# Autodesk Inventor assembly: circuittmp
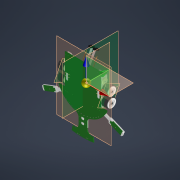
[picture p0: Inventor's stored thumbnail of the model, 180x180]
Saved by Autodesk Inventor 2022 (Build 260153000, 153)
## iProperties
Created: 2022-02-06
Part Number: circuittmp
Document SubType Name: Assembly
Designer: shiokaze
Author: shiokaze
## Documents named in this file (10)
- C:\Users\shiok\Documents\GitHub\murakumo\inventor\circuittmp.iam
- C:\Users\shiok\Documents\GitHub\murakumo\circuit\kicad\Step\Main.iam
- C:\Users\shiok\Documents\GitHub\murakumo\circuit\kicad\Step\Power.iam
- C:\Users\shiok\Documents\GitHub\murakumo\circuit\kicad\Step\SubSensor.iam
- C:\Users\shiok\Documents\GitHub\murakumo\circuit\kicad\Step\FrontSensor.iam
- C:\Users\shiok\Documents\GitHub\murakumo\inventor\Motor_MIR.iam
- C:\Users\shiok\Documents\GitHub\murakumo\inventor\jump.ipt
- C:\Users\shiok\Documents\GitHub\murakumo\inventor\SideSensorMount.ipt
- C:\Users\shiok\Documents\GitHub\murakumo\inventor\battery.ipt
- C:\Users\shiok\Documents\GitHub\murakumo\inventor\Motor_MIR_MIR.iam
## Components (11 placed, 9 different names)
1. Main:1 [sub-assembly] — メイト:1, メイト:2, メイト:3, メイト:10, 挿入:1, メイト:13, メイト:14, メイト:15, 角度:1, メイト:18, 挿入:2, メイト:25
2. Power:1 [sub-assembly] — メイト:4, メイト:5, メイト:6, 対称度:1, フラッシュ:1
3. SubSensor:2 [sub-assembly] — メイト:7, メイト:8, メイト:9
4. FrontSensor:1 [sub-assembly] — メイト:12, メイト:16, メイト:17
5. Motor_MIR:1 [sub-assembly] — メイト:1, メイト:2, メイト:3, メイト:4, メイト:5, メイト:6, 対称度:1, メイト:26
6. jump:1 — メイト:12, メイト:13, メイト:14, メイト:15, メイト:16, メイト:17
7. SideSensorMount:1 — メイト:7, メイト:8, メイト:9, メイト:10, 挿入:1
8. battery:1 — メイト:18, メイト:19, メイト:20
9. SideSensorMount:2 — メイト:21, メイト:22, メイト:23, 挿入:2
10. SubSensor:3 [sub-assembly] — メイト:21, メイト:22, メイト:23
11. Motor_MIR_MIR:1 [sub-assembly] — フラッシュ:2
## Relationships (31: Mate 25, Insert 2, Flush 2, Symmetry 1, Angle 1)
- メイト:1 [Mate]: Main:1 ↔ Motor_MIR:1
- メイト:2 [Mate]: Main:1 ↔ Motor_MIR:1
- メイト:3 [Mate]: Main:1 ↔ Motor_MIR:1
- メイト:4 [Mate]: Power:1 ↔ Motor_MIR:1
- メイト:5 [Mate]: Power:1 ↔ Motor_MIR:1
- メイト:6 [Mate]: Power:1 ↔ Motor_MIR:1
- 対称度:1 [Symmetry]: Power:1 ↔ Motor_MIR:1
- メイト:7 [Mate]: SubSensor:2 ↔ SideSensorMount:1
- メイト:8 [Mate]: SubSensor:2 ↔ SideSensorMount:1
- メイト:9 [Mate]: SubSensor:2 ↔ SideSensorMount:1
- メイト:10 [Mate]: Main:1 ↔ SideSensorMount:1
- 挿入:1 [Insert]: Main:1 ↔ SideSensorMount:1
- メイト:12 [Mate]: FrontSensor:1 ↔ jump:1
- メイト:13 [Mate]: Main:1 ↔ jump:1
- メイト:14 [Mate]: Main:1 ↔ jump:1
- メイト:15 [Mate]: Main:1 ↔ jump:1
- メイト:16 [Mate]: FrontSensor:1 ↔ jump:1
- メイト:17 [Mate]: FrontSensor:1 ↔ jump:1
- 角度:1 [Angle] (0 deg): Main:1
- メイト:18 [Mate]: Main:1 ↔ battery:1
- メイト:19 [Mate]: battery:1
- フラッシュ:1 [Flush] (-4.2 mm): Power:1
- メイト:20 [Mate]: battery:1
- メイト:21 [Mate]: SideSensorMount:2 ↔ SubSensor:3
- メイト:22 [Mate]: SideSensorMount:2 ↔ SubSensor:3
- メイト:23 [Mate]: SideSensorMount:2 ↔ SubSensor:3
- 挿入:2 [Insert]: Main:1 ↔ SideSensorMount:2
- メイト:24 [Mate]
- メイト:25 [Mate]: Main:1
- メイト:26 [Mate]: Motor_MIR:1
- フラッシュ:2 [Flush]: Motor_MIR_MIR:1
